# Autodesk Inventor assembly: Z-powertrain
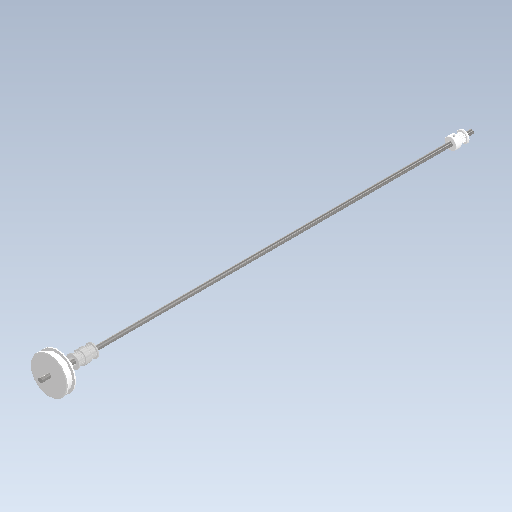
[picture p0: Inventor's stored thumbnail of the model, 512x512]
Saved by Autodesk Inventor 2020.4 (Build 244396000, 396)
## iProperties
Created: 2021-03-29
Part Number: Z-powertrain
Document SubType Name: Assembly
Designer: AOB
Mass: 139.116 g
Surface Area: 175.876 cm^2
Volume: 30.3292 cm^3
Density: 4.58686 g/cm^3
Author: AOB
## Documents named in this file (5)
- C:\Users\marti\Documents\Inventor\ProjectBoron\Boron Ultima\Z-powertrain.iam
- C:\Users\marti\Documents\Inventor\ProjectBoron\Boron Ultima\double-head pulley.ipt
- C:\Users\marti\Documents\Inventor\ProjectBoron\Boron Ultima\5mm shaft.ipt
- C:\Users\marti\Documents\Inventor\ProjectBoron\Boron Ultima\GT2 16T v2 (1) (1).ipt
- C:\Users\marti\Documents\Inventor\ProjectBoron\Boron Ultima\GT2 60T Pulley Powge.ipt
## Components (4 placed, 4 different names)
1. double-head pulley:1 — Mate:1, Mate:4
2. 5mm shaft:1 — Mate:1, Mate:2, Flush:1, Mate:3, Flush:2
3. GT2 16T v2 (1) (1):1 — Mate:2, Flush:1
4. GT2 60T Pulley Powge:1 — Mate:3, Flush:2, Mate:4
## Relationships (6: Mate 4, Flush 2)
- Mate:1: double-head pulley:1 ↔ 5mm shaft:1
- Mate:2: 5mm shaft:1 ↔ GT2 16T v2 (1) (1):1
- Flush:1 (9.5 mm): 5mm shaft:1 ↔ GT2 16T v2 (1) (1):1
- Mate:3: 5mm shaft:1 ↔ GT2 60T Pulley Powge:1
- Flush:2 (10 mm): 5mm shaft:1 ↔ GT2 60T Pulley Powge:1
- Mate:4 (10 mm): double-head pulley:1 ↔ GT2 60T Pulley Powge:1
